# Autodesk Inventor assembly: custom_chassis_MIR3
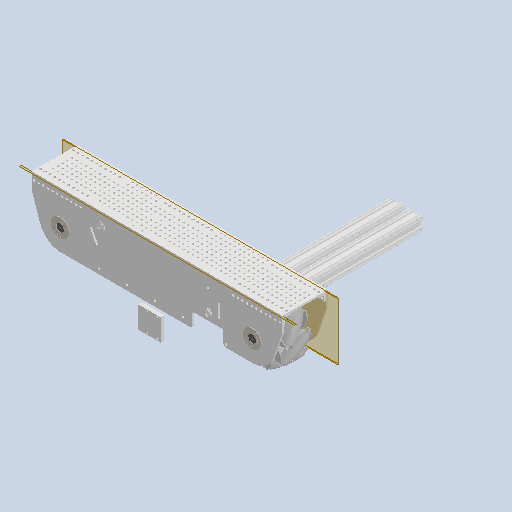
[picture p0: Inventor's stored thumbnail of the model, 512x512]
Saved by Autodesk Inventor 2022 (Build 260153000, 153)
## iProperties
Created: 2021-07-14
Part Number: custom_chassis_MIR3
Document SubType Name: Assembly
Designer: gfellows
Author: gfellows
## Documents named in this file (17)
- C:\Users\gfellows\Documents\GitHub\8103-CAD-2021-2022\custom_chassis_MIR3.iam
- C:\Users\gfellows\Documents\GitHub\8103-CAD-2021-2022\outside_plate_MIR3.ipt
- C:\Users\gfellows\Documents\GitHub\8103-CAD-2021-2022\100 mm mecanum wheel_MIR3.ipt
- C:\Users\gfellows\Documents\GitHub\8103-CAD-2021-2022\inside_plate_MIR3.ipt
- C:\Users\gfellows\Documents\GitHub\8103-CAD-2021-2022\1109-0024-0264_MIR3.ipt
- C:\Users\gfellows\Documents\GitHub\8103-CAD-2021-2022\am-3639 NeveRest Sport, 16-1 with Motor_MIR_MIR3.ipt
- C:\Users\gfellows\Documents\GitHub\8103-CAD-2021-2022\1611-0514-0006_MIR_MIR3.ipt
- C:\Users\gfellows\Documents\GitHub\8103-CAD-2021-2022\top_plate_MIR3.ipt
- C:\Users\gfellows\Documents\GitHub\8103-CAD-2021-2022\6mm axle for bevel gear and pulley_MIR3.ipt
- C:\Users\gfellows\Documents\GitHub\8103-CAD-2021-2022\0_500_Hex_ID_x_1_125_OD_x_0_313_WD_Flanged_Bearing_v2_217-3875 v1_MIR3.ipt
- C:\Users\gfellows\Documents\GitHub\8103-CAD-2021-2022\3417-1006-0016 assembly_MIR3.ipt
- C:\Users\gfellows\Documents\GitHub\8103-CAD-2021-2022\615398 assembly_MIR3.ipt
- C:\Users\gfellows\Documents\GitHub\8103-CAD-2021-2022\Axle for wheels 1_2_Hex_x_0_201_ID_ThunderHex_Stock_36_217-4017stp_MIR3.ipt
- C:\Users\gfellows\Documents\GitHub\8103-CAD-2021-2022\spacer_plate_MIR3.ipt
- C:\Users\gfellows\Documents\GitHub\8103-CAD-2021-2022\wheel_pulley_MIR3.ipt
- C:\Users\gfellows\Documents\GitHub\8103-CAD-2021-2022\1103-0011-0088_MIR3.ipt
- C:\Users\gfellows\Documents\GitHub\8103-CAD-2021-2022\2106-4008-0720 assembly_MIR3.ipt
## Components (41 placed, 16 different names)
1. outside_plate_MIR3:1
2. 100 mm mecanum wheel_MIR3:1
3. 100 mm mecanum wheel_MIR3:2
4. inside_plate_MIR3:1
5. 1109-0024-0264_MIR3:1
6. 1109-0024-0264_MIR3:2
7. am-3639 NeveRest Sport, 16-1 with Motor_MIR_MIR3:1
8. am-3639 NeveRest Sport, 16-1 with Motor_MIR_MIR3:2
9. 1611-0514-0006_MIR_MIR3:1
10. 1611-0514-0006_MIR_MIR3:2
11. 1611-0514-0006_MIR_MIR3:3
12. 1611-0514-0006_MIR_MIR3:4
13. top_plate_MIR3:1
14. 6mm axle for bevel gear and pulley_MIR3:1
15. 6mm axle for bevel gear and pulley_MIR3:2
16. 0_500_Hex_ID_x_1_125_OD_x_0_313_WD_Flanged_Bearing_v2_217-3875 v1_MIR3:1
17. 0_500_Hex_ID_x_1_125_OD_x_0_313_WD_Flanged_Bearing_v2_217-3875 v1_MIR3:2
18. 0_500_Hex_ID_x_1_125_OD_x_0_313_WD_Flanged_Bearing_v2_217-3875 v1_MIR3:3
19. 0_500_Hex_ID_x_1_125_OD_x_0_313_WD_Flanged_Bearing_v2_217-3875 v1_MIR3:4
20. 3417-1006-0016 assembly_MIR3:1
21. 3417-1006-0016 assembly_MIR3:2
22. 615398 assembly_MIR3:1
23. 615398 assembly_MIR3:2
24. 615398 assembly_MIR3:3
25. 615398 assembly_MIR3:4
26. Axle for wheels 1_2_Hex_x_0_201_ID_ThunderHex_Stock_36_217-4017stp_MIR3:1
27. Axle for wheels 1_2_Hex_x_0_201_ID_ThunderHex_Stock_36_217-4017stp_MIR3:2
28. spacer_plate_MIR3:1
29. wheel_pulley_MIR3:1
30. wheel_pulley_MIR3:2
31. 1103-0011-0088_MIR3:1
32. 1103-0011-0088_MIR3:2
33. 1103-0011-0088_MIR3:3
34. 2106-4008-0720 assembly_MIR3:1
35. 2106-4008-0720 assembly_MIR3:2
36. 2106-4008-0720 assembly_MIR3:3
37. 2106-4008-0720 assembly_MIR3:4
38. 2106-4008-0720 assembly_MIR3:5
39. 2106-4008-0720 assembly_MIR3:6
40. 1103-0011-0088_MIR3:4
41. 1103-0011-0088_MIR3:5
## Component patterns: (2 elements, first: 1103-0011-0088_MIR3:4)
